# Autodesk Inventor assembly: Mini-Circuits_BIAS-TEE_ZX85-12G-S+
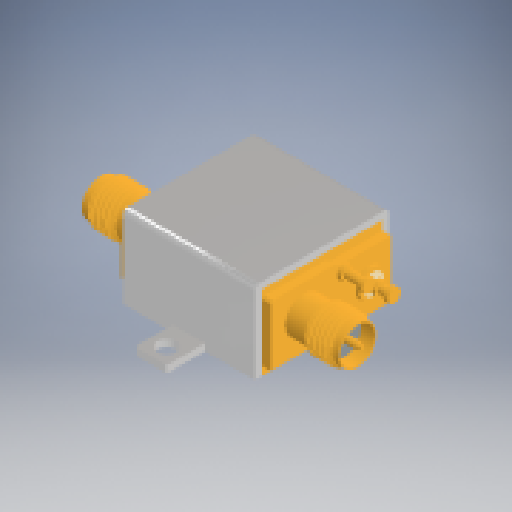
[picture p0: Inventor's stored thumbnail of the model, 512x512]
Saved by Autodesk Inventor 2025.2 (Build 292293000, 293)
## iProperties
Created: 2024-11-19
Part Number: Mini-Circuits_BIAS-TEE_ZX85-12G-S+
Document SubType Name: Assembly
Designer: Paul Linke
Author: Paul Linke
## Documents named in this file (3)
- C:\Users\PaulLinke\Documents\Inventor\MyLibrary\Assemblies\RF-Assemblies\Mini-Circuits_BIAS-TEE_ZX85-12G-S+.iam
- C:\Users\PaulLinke\Documents\Inventor\MyLibrary\Parts\RF-Parts\Mini-Circuits_Case_GC957.ipt
- C:\Users\PaulLinke\Documents\Inventor\MyLibrary\Parts\RF-Parts\SMA_PCB.ipt
## Components (3 placed, 2 different names)
1. Mini-Circuits_Case_GC957:1 — Planar:1, Mate:1, Mate:2, Planar:2, Mate:3, Mate:4
2. SMA_PCB:2 — Planar:1, Mate:1, Mate:2
3. SMA_PCB:1 — Planar:2, Mate:3, Mate:4
## Relationships (6: Mate 4, PlanarJoint 2)
- Planar:1: Mini-Circuits_Case_GC957:1 ↔ SMA_PCB:2
- Mate:1 (0.88 mm): Mini-Circuits_Case_GC957:1 ↔ SMA_PCB:2
- Mate:2: Mini-Circuits_Case_GC957:1 ↔ SMA_PCB:2
- Planar:2: Mini-Circuits_Case_GC957:1 ↔ SMA_PCB:1
- Mate:3: Mini-Circuits_Case_GC957:1 ↔ SMA_PCB:1
- Mate:4 (0.88 mm): Mini-Circuits_Case_GC957:1 ↔ SMA_PCB:1
